# Autodesk Inventor assembly: Assembly1
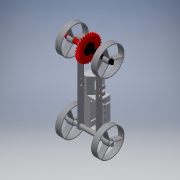
[picture p0: Inventor's stored thumbnail of the model, 180x180]
Saved by Autodesk Inventor 2018 (Build 220112000, 112)
## iProperties
Created: 2018-01-31
Part Number: Assembly1
Document SubType Name: Assembly
Designer: alber
Author: alber
## Documents named in this file (7)
- C:\Users\alber\OneDrive\Desktop\ENES100\CAD Assignment\Assembly\Assembly1.iam
- C:\Users\alber\OneDrive\Desktop\ENES100\CAD Assignment\Assembly\Motor Housing.ipt
- C:\Users\alber\OneDrive\Desktop\ENES100\CAD Assignment\Assembly\Sidewall.ipt
- C:\Users\alber\OneDrive\Desktop\ENES100\CAD Assignment\Assembly\Front Gear.ipt
- C:\Users\alber\OneDrive\Desktop\ENES100\CAD Assignment\Assembly\Front Axle.ipt
- C:\Users\alber\OneDrive\Desktop\ENES100\CAD Assignment\Assembly\Rear Axle.ipt
- C:\Users\alber\OneDrive\Desktop\ENES100\CAD Assignment\Assembly\Wheel.ipt
## Components (10 placed, 6 different names)
1. Motor Housing:1 — Mate:1, Mate:2, Mate:3, Mate:4
2. Sidewall:1 — Mate:2, Mate:3, Mate:4, Mate:5
3. Sidewall:2 — Mate:6, Mate:7
4. Front Gear:1 — Mate:5, Flush:1, Angle:1
5. Front Axle:1 — Mate:6, Flush:1, Angle:1, Flush:2, Angle:2
6. Rear Axle:1 — Mate:7, Flush:2, Angle:2, Mate:8, Mate:9, Angle:3, Mate:10
7. Wheel:1 — Mate:9, Angle:3, Mate:10
8. Wheel:2
9. Wheel:3
10. Wheel:4
## Component patterns: (4 elements, first: Wheel:1)
## Relationships (15: Mate 10, Angle 3, Flush 2)
- Mate:1: Motor Housing:1
- Mate:2: Motor Housing:1 ↔ Sidewall:1
- Mate:3 (0.5 mm): Motor Housing:1 ↔ Sidewall:1
- Mate:4 (0.35 mm): Motor Housing:1 ↔ Sidewall:1
- Mate:5: Sidewall:1 ↔ Front Gear:1
- Mate:6: Sidewall:2 ↔ Front Axle:1
- Flush:1: Front Gear:1 ↔ Front Axle:1
- Angle:1 (0 deg): Front Gear:1 ↔ Front Axle:1
- Mate:7: Sidewall:2 ↔ Rear Axle:1
- Flush:2: Front Axle:1 ↔ Rear Axle:1
- Angle:2 (0 deg): Front Axle:1 ↔ Rear Axle:1
- Mate:8 (-41.6 mm): Rear Axle:1
- Mate:9: Rear Axle:1 ↔ Wheel:1
- Angle:3 (180 deg): Rear Axle:1 ↔ Wheel:1
- Mate:10: Rear Axle:1 ↔ Wheel:1
